# Autodesk Inventor assembly: SampleHolder_1
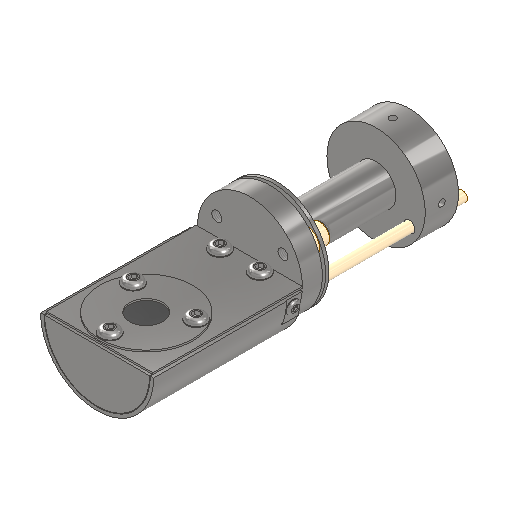
[picture p0: Inventor's stored thumbnail of the model, 512x512]
Saved by Autodesk Inventor 2026.2 (Build 302298000, 298)
## iProperties
Created: 2026-05-08
Part Number: SampleHolder_1
Document SubType Name: Assembly
Designer: zetsu
ProbePos: 738.000 mm
Author: zetsu
## Documents named in this file (16)
- D:\repos\PIHTI\BoronProbe_2026\SampleHolder_1.iam
- D:\repos\PIHTI\BoronProbe_2026\parts\B_holder_sub_5.ipt
- D:\repos\PIHTI\BoronProbe_2026\parts\M3x6-BHCS.ipt
- D:\repos\PIHTI\BoronProbe_2026\parts\ceramic_bushing_M3-v1.ipt
- D:\repos\PIHTI\BoronProbe_2026\parts\ceramic_washer_M4_v1.ipt
- D:\repos\PIHTI\BoronProbe_2026\parts\B_shield_5.iam
- D:\repos\PIHTI\BoronProbe_2026\parts\M2-4_screw.ipt
- D:\repos\PIHTI\BoronProbe_2026\parts\C25K22A4CU.iam
- D:\repos\PIHTI\BoronProbe_2026\parts\substrate.ipt
- D:\repos\PIHTI\BoronProbe_2026\parts\M3-nut.ipt
- D:\repos\PIHTI\BoronProbe_2026\parts\B_holder_up_5.ipt
- D:\repos\PIHTI\BoronProbe_2026\parts\M4×12-VentedHexBolt.ipt
- D:\repos\PIHTI\BoronProbe_2026\parts\B_probehead_5_1.ipt
- D:\repos\PIHTI\BoronProbe_2026\parts\B_pipe_cylinder_5_1.ipt
- D:\repos\PIHTI\BoronProbe_2026\parts\ceramic_2-hole-spacer_d3.ipt
- D:\repos\PIHTI\BoronProbe_2026\parts\ceramic_spacer_d3.ipt
## Components (36 placed, 15 different names)
1. B_probehead_5_1:1 — メイト:1, メイト:2, メイト:3, メイト:4, メイト:6, メイト:14, メイト:15, メイト:18, メイト:20, メイト:22, メイト:49, メイト:50, メイト:51, メイト:53, フラッシュ:2, メイト:54, フラッシュ:3, メイト:55, フラッシュ:4
2. B_holder_sub_5:1 — メイト:1, メイト:2, メイト:3, メイト:5, メイト:7, メイト:76, メイト:77, メイト:78, メイト:79, メイト:80, メイト:81, メイト:82, メイト:83, メイト:86
3. Broached Hexagon Socket Button Head Cap Screw - Metric M3 x 0.5 x 6:1 — メイト:4, メイト:5
4. Broached Hexagon Socket Button Head Cap Screw - Metric M3 x 0.5 x 6:2 — メイト:6, メイト:7
5. ceramic_bushing_M3-v1:2 — メイト:14, メイト:15, メイト:19
6. ceramic_washer_M4_v1:1 — メイト:20, メイト:43
7. ceramic_washer_M4_v1:2 — メイト:18, メイト:19, メイト:42
8. ceramic_washer_M4_v1:3 — メイト:22, メイト:44
9. B_pipe_cylinder_5_1:1 — メイト:42, メイト:43, メイト:44, メイト:93, メイト:94, メイト:95, メイト:96, メイト:97, メイト:98
10. B_shield_5:1 [sub-assembly] — メイト:49, メイト:50, メイト:51, メイト:56, メイト:57, メイト:58, メイト:59
11. ceramic_spacer_d3:1 — メイト:53, フラッシュ:2
12. ceramic_spacer_d3:2 — メイト:54, フラッシュ:3
13. ceramic_2-hole-spacer_d3:1 — メイト:55, フラッシュ:4
14. M2-4_screw:1 — メイト:56, メイト:57
15. M2-4_screw:2 — メイト:58, メイト:59
16. C25K22A4CU:1 [sub-assembly]
17. substrate:1 — メイト:76, メイト:77, メイト:84
18. JIS B 1181 Style 1 - Metric A M3:1 — メイト:78, メイト:79
19. JIS B 1181 Style 1 - Metric A M3:2 — メイト:82, メイト:83
20. JIS B 1181 Style 1 - Metric A M3:3 — メイト:80, メイト:81, メイト:85
21. B_holder_up_5:1 — メイト:84, メイト:85, メイト:86, メイト:87, メイト:88, メイト:89, メイト:90, メイト:91, メイト:92
22. Broached Hexagon Socket Button Head Cap Screw - Metric M3 x 0.5 x 6:8 — メイト:87, メイト:88
23. Broached Hexagon Socket Button Head Cap Screw - Metric M3 x 0.5 x 6:9 — メイト:89, メイト:90
24. Broached Hexagon Socket Button Head Cap Screw - Metric M3 x 0.5 x 6:10 — メイト:91, メイト:92
25. M4×12-VentedHexBolt:1
26. M4×12-VentedHexBolt:2
27. M4×12-VentedHexBolt:3
28. M4×12-VentedHexBolt:4
29. M4×12-VentedHexBolt:5
30. M4×12-VentedHexBolt:6
31. ceramic_bushing_M3-v1:4 — メイト:93, メイト:96, 挿入:1
32. Broached Hexagon Socket Button Head Cap Screw - Metric M3 x 0.5 x 6:11 — 挿入:1
33. ceramic_bushing_M3-v1:5 — メイト:94, メイト:97, 挿入:2
34. ceramic_bushing_M3-v1:6 — メイト:95, メイト:98, 挿入:3
35. Broached Hexagon Socket Button Head Cap Screw - Metric M3 x 0.5 x 6:12 — 挿入:3
36. Broached Hexagon Socket Button Head Cap Screw - Metric M3 x 0.5 x 6:13 — 挿入:2
## Relationships (55: Mate 49, Flush 3, Insert 3)
- メイト:1 [Mate]: B_probehead_5_1:1 ↔ B_holder_sub_5:1
- メイト:2 [Mate]: B_probehead_5_1:1 ↔ B_holder_sub_5:1
- メイト:3 [Mate]: B_probehead_5_1:1 ↔ B_holder_sub_5:1
- メイト:4 [Mate]: B_probehead_5_1:1 ↔ Broached Hexagon Socket Button Head Cap Screw - Metric M3 x 0.5 x 6:1
- メイト:5 [Mate]: B_holder_sub_5:1 ↔ Broached Hexagon Socket Button Head Cap Screw - Metric M3 x 0.5 x 6:1
- メイト:6 [Mate]: B_probehead_5_1:1 ↔ Broached Hexagon Socket Button Head Cap Screw - Metric M3 x 0.5 x 6:2
- メイト:7 [Mate]: B_holder_sub_5:1 ↔ Broached Hexagon Socket Button Head Cap Screw - Metric M3 x 0.5 x 6:2
- メイト:14 [Mate]: B_probehead_5_1:1 ↔ ceramic_bushing_M3-v1:2
- メイト:15 [Mate]: B_probehead_5_1:1 ↔ ceramic_bushing_M3-v1:2
- メイト:18 [Mate]: B_probehead_5_1:1 ↔ ceramic_washer_M4_v1:2
- メイト:19 [Mate]: ceramic_bushing_M3-v1:2 ↔ ceramic_washer_M4_v1:2
- メイト:20 [Mate]: B_probehead_5_1:1 ↔ ceramic_washer_M4_v1:1
- メイト:22 [Mate]: B_probehead_5_1:1 ↔ ceramic_washer_M4_v1:3
- メイト:42 [Mate]: ceramic_washer_M4_v1:2 ↔ B_pipe_cylinder_5_1:1
- メイト:43 [Mate]: ceramic_washer_M4_v1:1 ↔ B_pipe_cylinder_5_1:1
- メイト:44 [Mate]: ceramic_washer_M4_v1:3 ↔ B_pipe_cylinder_5_1:1
- メイト:49 [Mate]: B_probehead_5_1:1 ↔ B_shield_5:1
- メイト:50 [Mate]: B_probehead_5_1:1 ↔ B_shield_5:1
- メイト:51 [Mate]: B_probehead_5_1:1 ↔ B_shield_5:1
- メイト:53 [Mate]: B_probehead_5_1:1 ↔ ceramic_spacer_d3:1
- フラッシュ:2 [Flush]: B_probehead_5_1:1 ↔ ceramic_spacer_d3:1
- メイト:54 [Mate]: B_probehead_5_1:1 ↔ ceramic_spacer_d3:2
- フラッシュ:3 [Flush]: B_probehead_5_1:1 ↔ ceramic_spacer_d3:2
- メイト:55 [Mate]: B_probehead_5_1:1 ↔ ceramic_2-hole-spacer_d3:1
- フラッシュ:4 [Flush]: B_probehead_5_1:1 ↔ ceramic_2-hole-spacer_d3:1
- メイト:56 [Mate]: B_shield_5:1 ↔ M2-4_screw:1
- メイト:57 [Mate]: B_shield_5:1 ↔ M2-4_screw:1
- メイト:58 [Mate]: B_shield_5:1 ↔ M2-4_screw:2
- メイト:59 [Mate]: B_shield_5:1 ↔ M2-4_screw:2
- メイト:76 [Mate]: B_holder_sub_5:1 ↔ substrate:1
- メイト:77 [Mate]: B_holder_sub_5:1 ↔ substrate:1
- メイト:78 [Mate]: B_holder_sub_5:1 ↔ JIS B 1181 Style 1 - Metric A M3:1
- メイト:79 [Mate]: B_holder_sub_5:1 ↔ JIS B 1181 Style 1 - Metric A M3:1
- メイト:80 [Mate]: B_holder_sub_5:1 ↔ JIS B 1181 Style 1 - Metric A M3:3
- メイト:81 [Mate]: B_holder_sub_5:1 ↔ JIS B 1181 Style 1 - Metric A M3:3
- メイト:82 [Mate]: B_holder_sub_5:1 ↔ JIS B 1181 Style 1 - Metric A M3:2
- メイト:83 [Mate]: B_holder_sub_5:1 ↔ JIS B 1181 Style 1 - Metric A M3:2
- メイト:84 [Mate]: substrate:1 ↔ B_holder_up_5:1
- メイト:85 [Mate]: JIS B 1181 Style 1 - Metric A M3:3 ↔ B_holder_up_5:1
- メイト:86 [Mate]: B_holder_sub_5:1 ↔ B_holder_up_5:1
- メイト:87 [Mate]: B_holder_up_5:1 ↔ Broached Hexagon Socket Button Head Cap Screw - Metric M3 x 0.5 x 6:8
- メイト:88 [Mate]: B_holder_up_5:1 ↔ Broached Hexagon Socket Button Head Cap Screw - Metric M3 x 0.5 x 6:8
- メイト:89 [Mate]: B_holder_up_5:1 ↔ Broached Hexagon Socket Button Head Cap Screw - Metric M3 x 0.5 x 6:9
- メイト:90 [Mate]: B_holder_up_5:1 ↔ Broached Hexagon Socket Button Head Cap Screw - Metric M3 x 0.5 x 6:9
- メイト:91 [Mate]: B_holder_up_5:1 ↔ Broached Hexagon Socket Button Head Cap Screw - Metric M3 x 0.5 x 6:10
- メイト:92 [Mate]: B_holder_up_5:1 ↔ Broached Hexagon Socket Button Head Cap Screw - Metric M3 x 0.5 x 6:10
- メイト:93 [Mate]: B_pipe_cylinder_5_1:1 ↔ ceramic_bushing_M3-v1:4
- メイト:94 [Mate]: B_pipe_cylinder_5_1:1 ↔ ceramic_bushing_M3-v1:5
- メイト:95 [Mate]: B_pipe_cylinder_5_1:1 ↔ ceramic_bushing_M3-v1:6
- メイト:96 [Mate]: B_pipe_cylinder_5_1:1 ↔ ceramic_bushing_M3-v1:4
- メイト:97 [Mate]: B_pipe_cylinder_5_1:1 ↔ ceramic_bushing_M3-v1:5
- メイト:98 [Mate]: B_pipe_cylinder_5_1:1 ↔ ceramic_bushing_M3-v1:6
- 挿入:1 [Insert]: ceramic_bushing_M3-v1:4 ↔ Broached Hexagon Socket Button Head Cap Screw - Metric M3 x 0.5 x 6:11
- 挿入:2 [Insert]: ceramic_bushing_M3-v1:5 ↔ Broached Hexagon Socket Button Head Cap Screw - Metric M3 x 0.5 x 6:13
- 挿入:3 [Insert]: ceramic_bushing_M3-v1:6 ↔ Broached Hexagon Socket Button Head Cap Screw - Metric M3 x 0.5 x 6:12
## Named parameters: ProbePos = 738 mm, ProbePos_Max = 410 mm, ProbePos_Min = 738 mm
